# Autodesk Inventor assembly: ESC Encl
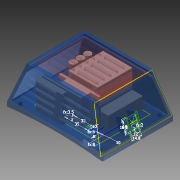
[picture p0: Inventor's stored thumbnail of the model, 180x180]
Saved by Autodesk Inventor 2015 SP1 (Build 190203100, 203)
## iProperties
Created: 2016-04-06
Part Number: ESC Encl
Document SubType Name: Assembly
Designer: doctor
Author: doctor
## Documents named in this file (5)
- C:\Users\dliu\Dropbox\dbhome\electric-longboard\dliu\EnclosureV2\ESC Encl.iam
- C:\Users\dliu\Dropbox\dbhome\electric-longboard\dliu\EnclosureV2\ESC Encl Bottom.ipt
- C:\Users\dliu\Dropbox\dbhome\electric-longboard\dliu\EnclosureV2\ESC Encl Lid.ipt
- C:\Users\dliu\Dropbox\dbhome\electric-longboard\dliu\Electronics\HobbyWing EZRUN 150A Pro 2.ipt
- C:\Users\dliu\Dropbox\dbhome\electric-longboard\dliu\EnclosureV2\TeensyBLENunchukBundle.ipt
## Components (4 placed, 4 different names)
1. ESC Encl Bottom:1 — Mate:1, Mate:2, Mate:3, Mate:5, Mate:6, Mate:7
2. ESC Encl Lid:1 — Mate:5, Mate:6, Mate:7
3. HobbyWing EZRUN 150A Pro 2:1 — Mate:1, Mate:3, Mate:4
4. TeensyBLENunchukBundle:1 — Mate:2, Mate:4
## Relationships (7: Mate 7)
- Mate:1: ESC Encl Bottom:1 ↔ HobbyWing EZRUN 150A Pro 2:1
- Mate:2: ESC Encl Bottom:1 ↔ TeensyBLENunchukBundle:1
- Mate:3: ESC Encl Bottom:1 ↔ HobbyWing EZRUN 150A Pro 2:1
- Mate:4 (2 mm): HobbyWing EZRUN 150A Pro 2:1 ↔ TeensyBLENunchukBundle:1
- Mate:5: ESC Encl Bottom:1 ↔ ESC Encl Lid:1
- Mate:6 (0.5 mm): ESC Encl Bottom:1 ↔ ESC Encl Lid:1
- Mate:7 (0.5 mm): ESC Encl Bottom:1 ↔ ESC Encl Lid:1
